# Autodesk Inventor assembly: yrail
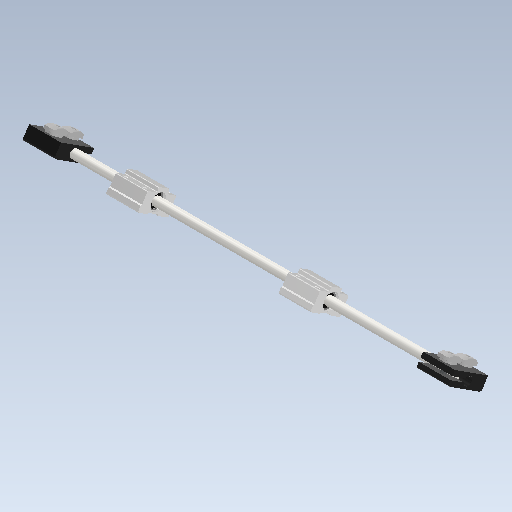
[picture p0: Inventor's stored thumbnail of the model, 512x512]
Saved by Autodesk Inventor 2020.2 (Build 242310000, 310)
## iProperties
Created: 2020-07-30
Part Number: yrail
Document SubType Name: Assembly
Designer: JK
Author: JK
## Documents named in this file (6)
- C:\Users\JK\Documents\Inventor\Anet Upgrade\yrail.iam
- C:\Users\JK\Documents\Inventor\Anet Upgrade\LinearBearing8mm.iam
- C:\Users\JK\Documents\Inventor\Anet Upgrade\8x380axis.ipt
- C:\Users\JK\Documents\Inventor\Anet Upgrade\yaxissupport.ipt
- C:\Users\JK\Documents\Inventor\Anet Upgrade\M5x15BoltFlatHead.ipt
- C:\Users\JK\Documents\Inventor\Anet Upgrade\T_Slot_Nut_Dropin_3030m5ipt.ipt
## Components (13 placed, 5 different names)
1. LinearBearing8mm:1 [sub-assembly]
2. LinearBearing8mm:2 [sub-assembly]
3. Wał:1
4. yaxissupport:1 — Mate:7, Mate:8, Mate:9, Angle:2, Mate:13, Angle:3
5. yaxissupport:2 — Mate:10, Mate:11, Angle:4, Mate:17
6. M5x15BoltFlatHead:1 — Mate:7, Mate:8, Flush:3, Flush:5, Mate:14
7. M5x15BoltFlatHead:2 — Mate:9, Flush:3, Mate:12
8. M5x15BoltFlatHead:3 — Mate:11, Flush:4, Mate:16
9. M5x15BoltFlatHead:4 — Mate:10, Flush:4, Flush:5, Mate:15
10. T_Slot_Nut_Dropin_3030m5ipt:1 — Mate:15, Flush:7, Flush:8
11. T_Slot_Nut_Dropin_3030m5ipt:2 — Mate:16, Angle:4, Flush:7, Mate:17, Flush:8
12. T_Slot_Nut_Dropin_3030m5ipt:3 — Mate:14, Flush:6, Angle:3
13. T_Slot_Nut_Dropin_3030m5ipt:4 — Mate:12, Angle:2, Mate:13, Flush:6
## Relationships (29: Mate 17, Flush 8, Angle 4)
- [Flush]: LinearBearing8mm:1 ↔ LinearBearing8mm:2
- [Mate]: LinearBearing8mm:1 ↔ LinearBearing8mm:2
- [Mate]: LinearBearing8mm:1 ↔ Wał:1
- [Mate]: Wał:1 ↔ yaxissupport:1
- [Mate] (0.5 mm): Wał:1 ↔ yaxissupport:1
- [Mate]: Wał:1 ↔ yaxissupport:2
- [Mate] (0.5 mm): Wał:1 ↔ yaxissupport:2
- [Flush]: yaxissupport:1 ↔ yaxissupport:2
- [Angle] (0 deg): LinearBearing8mm:1 ↔ yaxissupport:1
- Mate:7: yaxissupport:1 ↔ M5x15BoltFlatHead:1
- Mate:8: yaxissupport:1 ↔ M5x15BoltFlatHead:1
- Mate:9: yaxissupport:1 ↔ M5x15BoltFlatHead:2
- Flush:3: M5x15BoltFlatHead:1 ↔ M5x15BoltFlatHead:2
- Mate:10: yaxissupport:2 ↔ M5x15BoltFlatHead:4
- Mate:11: yaxissupport:2 ↔ M5x15BoltFlatHead:3
- Flush:4: M5x15BoltFlatHead:3 ↔ M5x15BoltFlatHead:4
- Flush:5: M5x15BoltFlatHead:1 ↔ M5x15BoltFlatHead:4
- Mate:12: M5x15BoltFlatHead:2 ↔ T_Slot_Nut_Dropin_3030m5ipt:4
- Angle:2 (0 deg): yaxissupport:1 ↔ T_Slot_Nut_Dropin_3030m5ipt:4
- Mate:13: yaxissupport:1 ↔ T_Slot_Nut_Dropin_3030m5ipt:4
- Mate:14: M5x15BoltFlatHead:1 ↔ T_Slot_Nut_Dropin_3030m5ipt:3
- Flush:6: T_Slot_Nut_Dropin_3030m5ipt:3 ↔ T_Slot_Nut_Dropin_3030m5ipt:4
- Angle:3 (0 deg): yaxissupport:1 ↔ T_Slot_Nut_Dropin_3030m5ipt:3
- Mate:15: M5x15BoltFlatHead:4 ↔ T_Slot_Nut_Dropin_3030m5ipt:1
- Mate:16: M5x15BoltFlatHead:3 ↔ T_Slot_Nut_Dropin_3030m5ipt:2
- Angle:4 (0 deg): yaxissupport:2 ↔ T_Slot_Nut_Dropin_3030m5ipt:2
- Flush:7: T_Slot_Nut_Dropin_3030m5ipt:1 ↔ T_Slot_Nut_Dropin_3030m5ipt:2
- Mate:17: yaxissupport:2 ↔ T_Slot_Nut_Dropin_3030m5ipt:2
- Flush:8: T_Slot_Nut_Dropin_3030m5ipt:1 ↔ T_Slot_Nut_Dropin_3030m5ipt:2
## Named parameters: d0_d2 = 0 mm, d1_d3 = 0 mm, d2_d4 = 0 mm, d3_d5 = 0 mm, d4_d6 = 0.5 mm, d5_d7 = 0 mm, d6_d8 = 0.5 mm
